# Autodesk Inventor assembly: KK8610P740A1F000_FILE_1
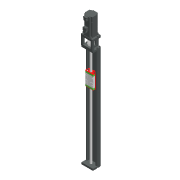
[picture p0: Inventor's stored thumbnail of the model, 180x180]
Saved by Autodesk Inventor 2021 (Build 250183000, 183)
## iProperties
Company: CADClick - www.CADClick.com
Created: 2021-08-22
Part Number: KK8610P740A1F000_FILE_1
Description: STEP AP214
Document SubType Name: Assembly
Designer: Santiago Suárez
Authority: unknown authorization
Title: cctmp_8B85085D-F73E-4B15-BE2D-5C7DA781C86F_2021_08_22_20_19_24_0268..stp
Author: HIWIN GmbH
Revision Number: NONE
Preprocessor: Spatial InterOp 3D
## Documents named in this file (5)
- C:\Users\Santiago Suárez\Documents\GitHub\Dis.-Mecatronico-E6\inventor proyecto\Guias\KK8610P740A1F000_FILE_1.iam
- C:\Users\Santiago Suárez\Documents\GitHub\Dis.-Mecatronico-E6\inventor proyecto\Guias\KK8610P740A1F000_FILE_1.ipt
- C:\Users\Santiago Suárez\Documents\GitHub\Dis.-Mecatronico-E6\inventor proyecto\Guias\KK8610P740A1F000_FILE.ipt
- C:\Users\Santiago Suárez\Documents\GitHub\Dis.-Mecatronico-E6\inventor proyecto\Guias\gsf_gr__2_d8_b___d14_b.ipt
- C:\Users\Santiago Suárez\Documents\GitHub\Dis.-Mecatronico-E6\inventor proyecto\Guias\MotorFRLS202B606A_FILE_2.ipt
## Components (4 placed, 4 different names)
1. KK8610P740A1F000_FILE_1 — Slider:1, Rigid:1
2. KK8610P740A1F000_FILE — Slider:1
3. gsf_gr__2_d8_b___d14_b:1 — Rigid:2
4. MotorFRLS202B606A_FILE_2:1 — Rigid:1, Rigid:2
## Relationships (3: WeldJoint 2, TranslationJoint 1)
- Slider:1 [TranslationJoint] (6 mm): KK8610P740A1F000_FILE_1 ↔ KK8610P740A1F000_FILE
- Rigid:1 [WeldJoint]: KK8610P740A1F000_FILE_1 ↔ MotorFRLS202B606A_FILE_2:1
- Rigid:2 [WeldJoint]: gsf_gr__2_d8_b___d14_b:1 ↔ MotorFRLS202B606A_FILE_2:1
